# Autodesk Inventor assembly: gakutasu-cat-wheel
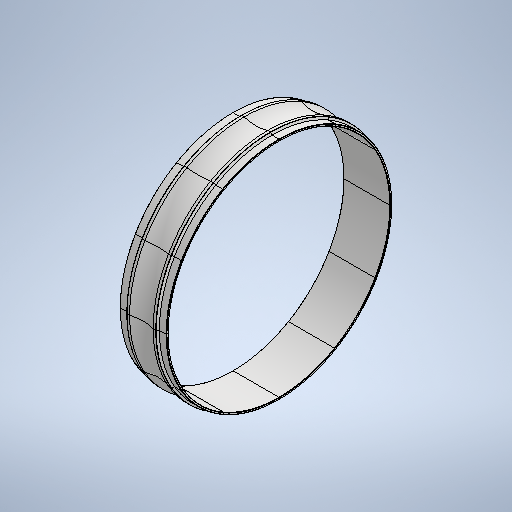
[picture p0: Inventor's stored thumbnail of the model, 512x512]
Saved by Autodesk Inventor 2026.2 (Build 302298000, 298)
## iProperties
Created: 2026-01-17
Part Number: gakutasu-cat-wheel
Document SubType Name: Assembly
Designer: gakut
Author: gakut
## Documents named in this file (3)
- C:\Users\gakut\Documents\Inventor\gakutasu-cat-wheel\gakutasu-cat-wheel.iam
- C:\Users\gakut\Documents\Inventor\gakutasu-cat-wheel\parts\wheel_plate.ipt
- C:\Users\gakut\Documents\Inventor\gakutasu-cat-wheel\parts\plate_joint_shaft.ipt
## Components (13 placed, 2 different names)
1. wheel_plate:1 — Rigid:1, Rigid:2
2. wheel_plate:2 — Rigid:2, Rigid:4
3. wheel_plate:3 — Rigid:4
4. wheel_plate:4 — Rigid:6
5. wheel_plate:5 — Rigid:6
6. wheel_plate:6 — Rigid:13
7. wheel_plate:7 — Rigid:13
8. wheel_plate:8
9. wheel_plate:9
10. wheel_plate:10
11. wheel_plate:11
12. wheel_plate:12
13. plate_joint_shaft:1 — Rigid:1
## Relationships (12: WeldJoint 12)
- Rigid:1 [WeldJoint]: wheel_plate:1 ↔ plate_joint_shaft:1
- Rigid:2 [WeldJoint]: wheel_plate:1 ↔ wheel_plate:2
- [WeldJoint]: wheel_plate:3 ↔ wheel_plate:4
- Rigid:4 [WeldJoint]: wheel_plate:2 ↔ wheel_plate:3
- [WeldJoint]: wheel_plate:5 ↔ wheel_plate:6
- Rigid:6 [WeldJoint]: wheel_plate:4 ↔ wheel_plate:5
- [WeldJoint]: wheel_plate:7 ↔ wheel_plate:8
- [WeldJoint]: wheel_plate:9 ↔ wheel_plate:10
- [WeldJoint]: wheel_plate:8 ↔ wheel_plate:9
- [WeldJoint]: wheel_plate:11 ↔ wheel_plate:12
- [WeldJoint]: wheel_plate:10 ↔ wheel_plate:11
- Rigid:13 [WeldJoint]: wheel_plate:6 ↔ wheel_plate:7
## Named parameters: d2_d1 = 0 mm, d4_d2_d1 = 0 mm, d7_d1 = 0 mm, d8_d2_d1 = 0 mm, d9_d3 = 0 mm, d10_d4_d2_d1 = 0 mm, d11_d5 = 0 mm
